# Autodesk Inventor assembly: IPT_track_assembly
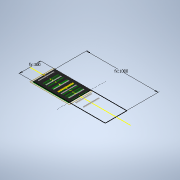
[picture p0: Inventor's stored thumbnail of the model, 180x180]
Saved by Autodesk Inventor 2020 (Build 240168000, 168)
## iProperties
Created: 2021-02-02
Part Number: IPT_track_assembly
Document SubType Name: Assembly
Designer: phamv
Author: phamv
## Documents named in this file (5)
- C:\Users\phamv\OneDrive\UoA\2020 SUMMER\2020-srw-rc-car\CoilDesign\DEXTER_WORKSPACE\CAD stuff\Final_CAD\IPT_track_assembly.iam
- C:\Users\phamv\OneDrive\UoA\2020 SUMMER\2020-srw-rc-car\CoilDesign\DEXTER_WORKSPACE\CAD stuff\Final_CAD\ferrite_layer_dex.ipt
- C:\Users\phamv\OneDrive\UoA\2020 SUMMER\2020-srw-rc-car\CoilDesign\DEXTER_WORKSPACE\CAD stuff\Final_CAD\spacer_0R2.ipt
- C:\Users\phamv\OneDrive\UoA\2020 SUMMER\2020-srw-rc-car\CoilDesign\DEXTER_WORKSPACE\CAD stuff\Final_CAD\ferrite_bar_long.ipt
- C:\Users\phamv\OneDrive\UoA\2020 SUMMER\2020-srw-rc-car\CoilDesign\DEXTER_WORKSPACE\CAD stuff\Final_CAD\bot_layer.ipt
## Components (10 placed, 4 different names)
1. ferrite_layer_dex:1 — Slider:1, Slider:2
2. bot_layer:1
3. spacer_0R2:1 — Slider:1
4. ferrite_bar_long:1 — Slider:2
5. ferrite_bar_long:2
6. ferrite_bar_long:3
7. ferrite_bar_long:4
8. ferrite_bar_long:5
9. ferrite_bar_long:6
10. ferrite_bar_long:7
## Component patterns: (7 elements, first: ferrite_bar_long:1)
## Relationships (2: TranslationJoint 2)
- Slider:1 [TranslationJoint]: ferrite_layer_dex:1 ↔ spacer_0R2:1
- Slider:2 [TranslationJoint]: ferrite_layer_dex:1 ↔ ferrite_bar_long:1
